# Autodesk Inventor assembly: assembly_fp16
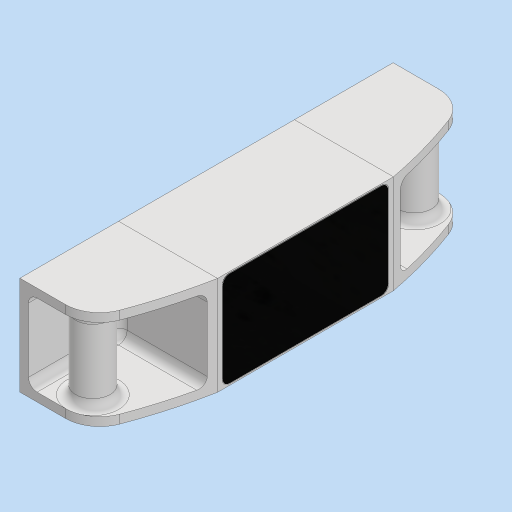
[picture p0: Inventor's stored thumbnail of the model, 512x512]
Saved by Autodesk Inventor 2023 (Build 270158000, 158)
## iProperties
Created: 2023-04-11
Part Number: assembly_fp16
Document SubType Name: Assembly
Designer: tdal0
Author: tdal0
## Documents named in this file (4)
- C:\4806\front panel parts\assembly_fp16.iam
- C:\4806\front panel parts\center_fp16.ipt
- C:\4806\front panel parts\sides_fp15.ipt
- C:\4806\front panel parts\raspberry pi display.iam
## Components (4 placed, 3 different names)
1. center_fp16:1 — Flush:1, Mate:1, Mate:2, Flush:2, Mate:3, Mate:4, Mate:5, Mate:6, Flush:3
2. sides_fp15:1 — Flush:1, Mate:1, Mate:2
3. sides_fp15:2 — Flush:2, Mate:3, Mate:4
4. raspberry pi display:1 [sub-assembly] — Mate:5, Mate:6, Flush:3
## Relationships (9: Mate 6, Flush 3)
- Flush:1: center_fp16:1 ↔ sides_fp15:1
- Mate:1: center_fp16:1 ↔ sides_fp15:1
- Mate:2: center_fp16:1 ↔ sides_fp15:1
- Flush:2: center_fp16:1 ↔ sides_fp15:2
- Mate:3: center_fp16:1 ↔ sides_fp15:2
- Mate:4: center_fp16:1 ↔ sides_fp15:2
- Mate:5: center_fp16:1 ↔ raspberry pi display:1
- Mate:6: center_fp16:1 ↔ raspberry pi display:1
- Flush:3: center_fp16:1 ↔ raspberry pi display:1
